# Autodesk Inventor assembly: moulding_assembly_stage2
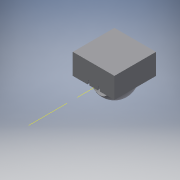
[picture p0: Inventor's stored thumbnail of the model, 180x180]
Saved by Autodesk Inventor 2017 (Build 210142000, 142)
## iProperties
Created: 2018-06-01
Part Number: moulding_assembly_stage2
Document SubType Name: Assembly
Designer: Nic
Author: Nic
## Documents named in this file (3)
- C:\Users\Nic\Documents\Antenna\moulding_assembly_stage2.iam
- C:\Users\Nic\Documents\Antenna\mould-stage-1.ipt
- C:\Users\Nic\Documents\Antenna\sensor_pad.ipt
## Components (2 placed, 2 different names)
1. sensor_pad:1 — Mate:1, Mate:2
2. mould-stage-1:1 — Mate:2, Mate:3
## Relationships (3: Mate 3)
- Mate:1: sensor_pad:1
- Mate:2: sensor_pad:1 ↔ mould-stage-1:1
- Mate:3: mould-stage-1:1
